# Autodesk Inventor assembly: Full overlay hinge for aluminium frame
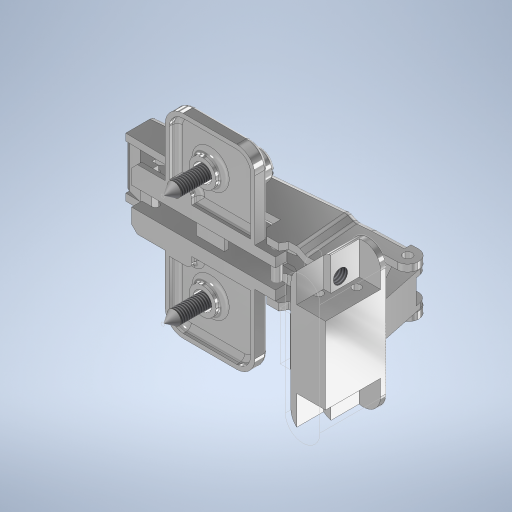
[picture p0: Inventor's stored thumbnail of the model, 512x512]
Saved by Autodesk Inventor 2024 (Build 280153000, 153)
## iProperties
Created: 2014-01-06
Part Number: Full overlay hinge for aluminium frame
Document SubType Name: Assembly
Designer: G. Kazokaitis
Author: G. Kazokaitis
## Documents named in this file (7)
- C:\W4INV 2024 Design\_LIBRARY\Hinges\HINGE FOR ALUMINIUM FRAME\Full overlay hinge for aluminium frame.iam
- C:\W4INV 2024 Design\LIBRARY\Hinges\Parts\Hinge for aluminium frame\Full overlay case .ipt
- C:\W4INV 2024 Design\LIBRARY\Hinges\Parts\Hinge for aluminium frame\Lever for full overlay hinge.ipt
- C:\W4INV 2024 Design\LIBRARY\Hinges\Parts\Hinge for aluminium frame\Linkage for full overlay hinge.ipt
- C:\W4INV 2024 Design\LIBRARY\Hinges\Parts\Hinge for aluminium frame\Mounting plate.ipt
- C:\W4INV 2024 Design\LIBRARY\Hinges\Parts\Hinge for aluminium frame\Cup.ipt
- C:\W4INV 2024 Design\LIBRARY\Hinges\HINGE FOR ALUMINIUM FRAME.iam
## Components (5 placed, 5 different names)
1. Mounting plate:1 — Flush:1, Flush:2, Mate:1, Flush:3, Mate:2, Mate:3
2. Cup:1 — Mate:8, Mate:9, Mate:10, Full overlay opening angle
3. Full overlay case :1 — Flush:3, Mate:2, Mate:3, Mate:4, Mate:5, Mate:6, Mate:7, Full overlay opening angle
4. Linkage for full overlay hinge:1 — Mate:5, Mate:7, Mate:9
5. Lever for full overlay hinge:1 — Mate:4, Mate:6, Mate:8, Mate:10
## Relationships (14: Mate 10, Flush 3, Angle 1)
- Flush:1: Mounting plate:1
- Flush:2: Mounting plate:1
- Mate:1: Mounting plate:1
- Flush:3: Mounting plate:1 ↔ Full overlay case :1
- Mate:2: Mounting plate:1 ↔ Full overlay case :1
- Mate:3: Mounting plate:1 ↔ Full overlay case :1
- Mate:4: Full overlay case :1 ↔ Lever for full overlay hinge:1
- Mate:5: Full overlay case :1 ↔ Linkage for full overlay hinge:1
- Mate:6 (0.2 mm): Full overlay case :1 ↔ Lever for full overlay hinge:1
- Mate:7 (0.2 mm): Full overlay case :1 ↔ Linkage for full overlay hinge:1
- Mate:8: Cup:1 ↔ Lever for full overlay hinge:1
- Mate:9: Cup:1 ↔ Linkage for full overlay hinge:1
- Mate:10 (1.9 mm): Cup:1 ↔ Lever for full overlay hinge:1
- Full overlay opening angle [Angle] (180 deg): Cup:1 ↔ Full overlay case :1
## Named parameters: Offset_distance = 37 mm
